# Autodesk Inventor assembly: byk_alternator
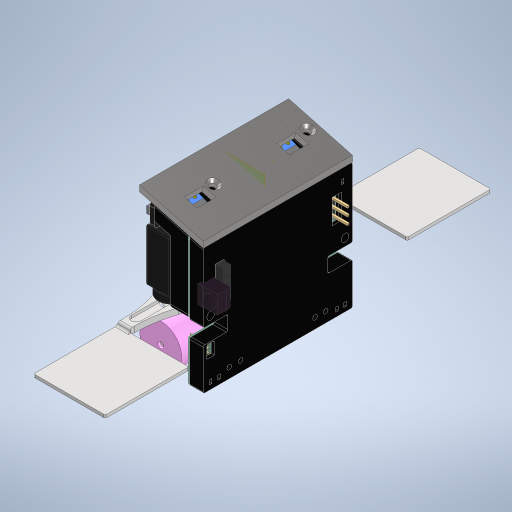
[picture p0: Inventor's stored thumbnail of the model, 512x512]
Saved by Autodesk Inventor 2023 (Build 270158000, 158)
## iProperties
Created: 2023-12-19
Part Number: byk_alternator
Document SubType Name: Assembly
Designer: Kamil
Author: Kamil
## Documents named in this file (12)
- C:\Users\kamil\Documents\PROJECTS - repos\Stratos---MicroSumo\mechanics\byk_alternator.iam
- C:\Users\kamil\Documents\PROJECTS - repos\Stratos---MicroSumo\mechanics\servo_mini_1370hd_cos.ipt
- C:\Users\kamil\Documents\PROJECTS - repos\Stratos---MicroSumo\mechanics\podstawa.ipt
- C:\Users\kamil\Documents\PROJECTS - repos\Stratos---MicroSumo\mechanics\noz2.ipt
- C:\Users\kamil\Documents\PROJECTS - repos\Stratos---MicroSumo\mechanics\QRE1113GR.ipt
- C:\Users\kamil\Documents\PROJECTS - repos\Stratos---MicroSumo\mechanics\silnik_2.ipt
- C:\Users\kamil\Documents\PROJECTS - repos\Stratos---MicroSumo\mechanics\kolko.ipt
- C:\Users\kamil\Documents\PROJECTS - repos\Stratos---MicroSumo\mechanics\pcb_dolne.ipt
- C:\Users\kamil\Documents\PROJECTS - repos\Stratos---MicroSumo\mechanics\30x20x5.ipt
- C:\Users\kamil\Documents\PROJECTS - repos\Stratos---MicroSumo\mechanics\MikroSumo.ipt
- C:\Users\kamil\Documents\PROJECTS - repos\Stratos---MicroSumo\mechanics\dach.ipt
- C:\Users\kamil\Documents\PROJECTS - repos\Stratos---MicroSumo\mechanics\wachlarz.ipt
## Components (16 placed, 11 different names)
1. servo_mini_1370hd_cos:1 — Zestawiające:1, Równoległe:1, Równoległe:2, Zestawiające:57, Zestawiające:58
2. servo_mini_1370hd_cos:2 — Zestawiające:1, Równoległe:1, Równoległe:2, Równoległe:3, Zestawiające:55, Zestawiające:56
3. podstawa:1 — Równoległe:3, Równoległe:4, Zestawiające:11, Równoległe:5, Równoległe:6, Zestawiające:17, Zestawiające:18, Zestawiające:19, Równoległe:7, Zestawiające:20, Zestawiające:38, Zestawiające:39, Zestawiające:46, Zestawiające:47, Zestawiające:48, Zestawiające:49, Zestawiające:50, Zestawiające:51
4. noz2:1 — Równoległe:4
5. QRE1113GR:1 — Zestawiające:18
6. QRE1113GR:2 — Zestawiające:17
7. silnik_2:1 — Zestawiające:11, Zestawiające:12, Zestawiające:13, Zestawiające:16
8. silnik_2:2 — Zestawiające:12, Zestawiające:13, Zestawiające:14, Zestawiające:15
9. kolko:1 — Zestawiające:14, Zestawiające:15, Równoległe:5
10. kolko:2 — Równoległe:6, Zestawiające:16
11. pcb_dolne:1 — Zestawiające:19, Równoległe:7, Zestawiające:20
12. 30x20x5:1 — Zestawiające:38, Zestawiające:39, Zestawiające:46, Zestawiające:47, Zestawiające:48
13. MikroSumo:2 — Zestawiające:49, Zestawiające:50, Zestawiające:51, Zestawiające:52, Zestawiające:53, Zestawiające:54
14. dach:1 — Zestawiające:52, Zestawiające:53, Zestawiające:54
15. wachlarz:1 — Zestawiające:55, Zestawiające:56, Kątowe:1, Równoległe:8
16. wachlarz:2 — Zestawiające:57, Zestawiające:58, Kątowe:1, Równoległe:8
## Relationships (35: Mate 26, Flush 8, Angle 1)
- Zestawiające:1 [Mate] (-50 mm): servo_mini_1370hd_cos:1 ↔ servo_mini_1370hd_cos:2
- Równoległe:1 [Flush]: servo_mini_1370hd_cos:1 ↔ servo_mini_1370hd_cos:2
- Równoległe:2 [Flush]: servo_mini_1370hd_cos:1 ↔ servo_mini_1370hd_cos:2
- Równoległe:3 [Flush]: servo_mini_1370hd_cos:2 ↔ podstawa:1
- Równoległe:4 [Flush]: podstawa:1 ↔ noz2:1
- Zestawiające:11 [Mate]: podstawa:1 ↔ silnik_2:1
- Zestawiające:12 [Mate] (2 mm): silnik_2:1 ↔ silnik_2:2
- Zestawiające:13 [Mate]: silnik_2:1 ↔ silnik_2:2
- Zestawiające:14 [Mate]: silnik_2:2 ↔ kolko:1
- Zestawiające:15 [Mate]: silnik_2:2 ↔ kolko:1
- Równoległe:5 [Flush]: podstawa:1 ↔ kolko:1
- Równoległe:6 [Flush]: podstawa:1 ↔ kolko:2
- Zestawiające:16 [Mate]: silnik_2:1 ↔ kolko:2
- Zestawiające:17 [Mate] (1.6 mm): podstawa:1 ↔ QRE1113GR:2
- Zestawiające:18 [Mate] (1.6 mm): podstawa:1 ↔ QRE1113GR:1
- Zestawiające:19 [Mate]: podstawa:1 ↔ pcb_dolne:1
- Równoległe:7 [Flush]: podstawa:1 ↔ pcb_dolne:1
- Zestawiające:20 [Mate]: podstawa:1 ↔ pcb_dolne:1
- Zestawiające:38 [Mate]: podstawa:1 ↔ 30x20x5:1
- Zestawiające:39 [Mate] (0.1 mm): podstawa:1 ↔ 30x20x5:1
- Zestawiające:46 [Mate]: podstawa:1 ↔ 30x20x5:1
- Zestawiające:47 [Mate]: podstawa:1 ↔ 30x20x5:1
- Zestawiające:48 [Mate]: podstawa:1 ↔ 30x20x5:1
- Zestawiające:49 [Mate]: podstawa:1 ↔ MikroSumo:2
- Zestawiające:50 [Mate]: podstawa:1 ↔ MikroSumo:2
- Zestawiające:51 [Mate]: podstawa:1 ↔ MikroSumo:2
- Zestawiające:52 [Mate]: MikroSumo:2 ↔ dach:1
- Zestawiające:53 [Mate]: MikroSumo:2 ↔ dach:1
- Zestawiające:54 [Mate]: MikroSumo:2 ↔ dach:1
- Zestawiające:55 [Mate] (1 mm): servo_mini_1370hd_cos:2 ↔ wachlarz:1
- Zestawiające:56 [Mate]: servo_mini_1370hd_cos:2 ↔ wachlarz:1
- Zestawiające:57 [Mate] (1 mm): servo_mini_1370hd_cos:1 ↔ wachlarz:2
- Zestawiające:58 [Mate]: servo_mini_1370hd_cos:1 ↔ wachlarz:2
- Kątowe:1 [Angle] (0 deg): wachlarz:1 ↔ wachlarz:2
- Równoległe:8 [Flush]: wachlarz:1 ↔ wachlarz:2
